# Autodesk Inventor assembly: Enclosure02
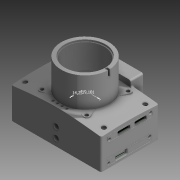
[picture p0: Inventor's stored thumbnail of the model, 180x180]
Saved by Autodesk Inventor 2013 (Build 170138000, 138)
## iProperties
Created: 2014-04-13
Part Number: Enclosure02
Document SubType Name: Assembly
Designer: spichelh
Author: spichelh
## Documents named in this file (17)
- C:\Users\spichelh\Documents\GitHub\beta-hardware\Enclosure\Version 002\Enclosure02.iam
- C:\Users\spichelh\Documents\GitHub\beta-hardware\Enclosure\Version 002\PCB01.ipt
- C:\Users\spichelh\Documents\GitHub\beta-hardware\Enclosure\Version 002\Microzed01.ipt
- C:\Users\spichelh\Documents\GitHub\beta-hardware\Enclosure\Version 002\AddonPCB01.ipt
- C:\Users\spichelh\Documents\GitHub\beta-hardware\Enclosure\Version 002\Enclosure-Backplate01.ipt
- C:\Users\spichelh\Documents\GitHub\beta-hardware\Enclosure\Version 002\KAC12040.ipt
- C:\Users\spichelh\Documents\GitHub\beta-hardware\Enclosure\Version 002\IRGlass.ipt
- C:\Users\spichelh\Documents\GitHub\beta-hardware\Enclosure\Version 002\Cooler.ipt
- C:\Users\spichelh\Documents\GitHub\beta-hardware\Enclosure\Version 002\Enclosure02.ipt
- C:\Users\spichelh\Documents\GitHub\beta-hardware\Enclosure\Version 002\Nikon Mount 02.ipt
- C:\Users\spichelh\Documents\GitHub\beta-hardware\Enclosure\Version 002\IOModulePlate01.ipt
- C:\Users\spichelh\Documents\GitHub\beta-hardware\Enclosure\Version 002\PCBModuleLeft01.ipt
- C:\Users\spichelh\Documents\GitHub\beta-hardware\Enclosure\Version 002\IOModulePlate02.ipt
- C:\Users\spichelh\Documents\GitHub\beta-hardware\Enclosure\Version 002\IOModulePlate03.ipt
- C:\Users\spichelh\Documents\GitHub\beta-hardware\Enclosure\Version 002\PCBModuleRight01.ipt
- C:\Users\spichelh\Documents\GitHub\beta-hardware\Enclosure\Version 002\LensBase02.ipt
- C:\Users\spichelh\Documents\GitHub\beta-hardware\Enclosure\Version 002\HexSaver01.ipt
## Components (19 placed, 16 different names)
1. Enclosure02:1 — Flush:26, Mate:33, Mate:34, Mate:38, Flush:39, Flush:40, Mate:39, Insert:9, Insert:10, Insert:11, Insert:12, Insert:13, Insert:14
2. PCB01:1 — Mate:1, Flush:1, Flush:2, Mate:30, Flush:21, Flush:22, Flush:23, Insert:1, Mate:37, Flush:41, Flush:42, Mate:40, Mate:41, Mate:42, Mate:43, Mate:44, Mate:45, Insert:15, Mate:46, Mate:47, Insert:16, Mate:48, Mate:49, Insert:17
3. Microzed01:1 — Mate:1, Flush:1, Flush:2, Flush:22, Flush:24, Flush:27, Mate:36
4. AddonPCB01:1 — Flush:24, Flush:27, Mate:36
5. Enclosure-Backplate01:1 — Mate:38, Flush:39, Flush:40
6. KAC12040:1 — Mate:37
7. IRGlass:1 — Mate:50, Mate:51, Mate:52
8. Cooler:1 — Mate:35
9. Nikon Mount 02:1 — Mate:31, Mate:32, Insert:3, Mate:50, Mate:51, Mate:52
10. LensBase02:1 — Mate:31, Mate:32, Insert:1, Flush:26, Mate:33, Mate:34, Insert:3, Mate:35
11. IOModulePlate01:1 — Insert:13, Insert:14
12. PCBModuleLeft01:1 — Mate:30, Flush:21, Flush:23
13. PCBModuleRight01:1 — Flush:41, Flush:42, Mate:40
14. IOModulePlate02:1 — Insert:11, Insert:12
15. IOModulePlate03:1 — Insert:9, Insert:10
16. HexSaver01:1 — Mate:41, Mate:42, Mate:43
17. HexSaver01:2 — Mate:44, Mate:45, Insert:15
18. HexSaver01:3 — Mate:46, Mate:47, Insert:16
19. HexSaver01:4 — Mate:48, Mate:49, Insert:17
## Relationships (47: Mate 24, Flush 12, Insert 11)
- Mate:1 (5 mm): PCB01:1 ↔ Microzed01:1
- Flush:1: PCB01:1 ↔ Microzed01:1
- Flush:2: PCB01:1 ↔ Microzed01:1
- Mate:30 (6 mm): PCB01:1 ↔ PCBModuleLeft01:1
- Flush:21: PCB01:1 ↔ PCBModuleLeft01:1
- Flush:22: PCB01:1 ↔ Microzed01:1
- Flush:23: PCB01:1 ↔ PCBModuleLeft01:1
- Flush:24: Microzed01:1 ↔ AddonPCB01:1
- Mate:31: Nikon Mount 02:1 ↔ LensBase02:1
- Mate:32: Nikon Mount 02:1 ↔ LensBase02:1
- Insert:1: PCB01:1 ↔ LensBase02:1
- Flush:26: Enclosure02:1 ↔ LensBase02:1
- Mate:33: Enclosure02:1 ↔ LensBase02:1
- Mate:34: Enclosure02:1 ↔ LensBase02:1
- Insert:3: Nikon Mount 02:1 ↔ LensBase02:1
- Mate:35: Cooler:1 ↔ LensBase02:1
- Flush:27: Microzed01:1 ↔ AddonPCB01:1
- Mate:36 (10 mm): Microzed01:1 ↔ AddonPCB01:1
- Mate:37: PCB01:1 ↔ KAC12040:1
- Mate:38 (-1 mm): Enclosure02:1 ↔ Enclosure-Backplate01:1
- Flush:39: Enclosure02:1 ↔ Enclosure-Backplate01:1
- Flush:40: Enclosure02:1 ↔ Enclosure-Backplate01:1
- Mate:39: Enclosure02:1
- Flush:41: PCB01:1 ↔ PCBModuleRight01:1
- Flush:42: PCB01:1 ↔ PCBModuleRight01:1
- Mate:40 (6 mm): PCB01:1 ↔ PCBModuleRight01:1
- Insert:9: Enclosure02:1 ↔ IOModulePlate03:1
- Insert:10: Enclosure02:1 ↔ IOModulePlate03:1
- Insert:11: Enclosure02:1 ↔ IOModulePlate02:1
- Insert:12: Enclosure02:1 ↔ IOModulePlate02:1
- Insert:13: Enclosure02:1 ↔ IOModulePlate01:1
- Insert:14: Enclosure02:1 ↔ IOModulePlate01:1
- Mate:41: PCB01:1 ↔ HexSaver01:1
- Mate:42: PCB01:1 ↔ HexSaver01:1
- Mate:43: PCB01:1 ↔ HexSaver01:1
- Mate:44: PCB01:1 ↔ HexSaver01:2
- Mate:45: PCB01:1 ↔ HexSaver01:2
- Insert:15: PCB01:1 ↔ HexSaver01:2
- Mate:46: PCB01:1 ↔ HexSaver01:3
- Mate:47: PCB01:1 ↔ HexSaver01:3
- Insert:16: PCB01:1 ↔ HexSaver01:3
- Mate:48: PCB01:1 ↔ HexSaver01:4
- Mate:49: PCB01:1 ↔ HexSaver01:4
- Insert:17: PCB01:1 ↔ HexSaver01:4
- Mate:50: IRGlass:1 ↔ Nikon Mount 02:1
- Mate:51 (0.5 mm): IRGlass:1 ↔ Nikon Mount 02:1
- Mate:52 (0.5 mm): IRGlass:1 ↔ Nikon Mount 02:1
